# Autodesk Inventor assembly: Shipping goods QR subassembly 1 roq
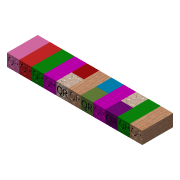
[picture p0: Inventor's stored thumbnail of the model, 180x180]
Saved by Autodesk Inventor 2015 (Build 190159000, 159)
## iProperties
Created: 2015-03-08
Part Number: Shipping goods QR subassembly 1 roq
Document SubType Name: Assembly
Designer: Vukica
Author: Vukica
## Documents named in this file (12)
- C:\Users\Vukica\Dropbox\IEEE\hardware rules\2016Hardware_Court_v6\Shipping goods QR subassembly 1 roq.iam
- C:\Users\Vukica\Dropbox\IEEE\hardware rules\2016Hardware_Court_v6\Container 2 2 5.ipt
- C:\Users\Vukica\Dropbox\IEEE\hardware rules\2016Hardware_Court_v6\Container 2 2 2 and half.ipt
- C:\Users\Vukica\Dropbox\IEEE\hardware rules\2016Hardware_Court_v6\Container 2 2 2 and half color 2.ipt
- C:\Users\Vukica\Dropbox\IEEE\hardware rules\2016Hardware_Court_v6\Container 2 2 2 and half color 4.ipt
- C:\Users\Vukica\Dropbox\IEEE\hardware rules\2016Hardware_Court_v6\Container 2 2 2 and half color 5.ipt
- C:\Users\Vukica\Dropbox\IEEE\hardware rules\2016Hardware_Court_v6\Container 2 2 2 and half color 7.ipt
- C:\Users\Vukica\Dropbox\IEEE\hardware rules\2016Hardware_Court_v6\Container 2 2 5 QR color 4.ipt
- C:\Users\Vukica\Dropbox\IEEE\hardware rules\2016Hardware_Court_v6\Container 2 2 5 QR color 5.ipt
- C:\Users\Vukica\Dropbox\IEEE\hardware rules\2016Hardware_Court_v6\Container 2 2 5 QR color 6.ipt
- C:\Users\Vukica\Dropbox\IEEE\hardware rules\2016Hardware_Court_v6\Container 2 2 5 QR color 1.ipt
- C:\Users\Vukica\Dropbox\IEEE\hardware rules\2016Hardware_Court_v6\Container 2 2 5 QR color 2.ipt
## Components (14 placed, 11 different names)
1. Container 2 2 5:1 — Flush:1, Mate:1, Flush:2, Flush:4, Mate:4, Flush:6, Flush:8
2. Container 2 2 2 and half:1 — Flush:1, Mate:1, Flush:2, Flush:3, Mate:2, Mate:8
3. Container 2 2 2 and half color 2:1 — Flush:5, Mate:3, Flush:7, Mate:5, Flush:9, Flush:10, Mate:9
4. Container 2 2 2 and half color 4:1 — Mate:7, Mate:8, Flush:13
5. Container 2 2 2 and half color 5:1 — Mate:9, Mate:10, Flush:14
6. Container 2 2 2 and half color 7:1 — Mate:13, Flush:19, Flush:20, Mate:14, Flush:21, Flush:22, Flush:23, Mate:32, Flush:56, Flush:57
7. Container 2 2 5 QR color 4:1 — Flush:3, Mate:2, Flush:4, Flush:5, Mate:3, Flush:7, Mate:7, Flush:13, Mate:10, Flush:14
8. Container 2 2 5 QR color 5:1 — Mate:6, Flush:11, Flush:12, Mate:11, Flush:15, Flush:16
9. Container 2 2 5 QR color 6:1 — Mate:11, Flush:15, Flush:16
10. Container 2 2 5 QR color 1:1 — Mate:5, Flush:9, Flush:10, Mate:13, Flush:19, Flush:20
11. Container 2 2 5 QR color 2:1 — Mate:4, Flush:6, Flush:8, Mate:6, Flush:11, Flush:12
12. Container 2 2 2 and half:2 — Mate:14, Flush:21, Flush:22, Flush:23
13. Container 2 2 5 QR color 2:4 — Mate:32, Flush:56, Flush:57, Mate:33, Flush:58, Flush:59
14. Container 2 2 5 QR color 4:3 — Mate:33, Flush:58, Flush:59
## Relationships (40: Flush 25, Mate 15)
- Flush:1: Container 2 2 5:1 ↔ Container 2 2 2 and half:1
- Mate:1: Container 2 2 5:1 ↔ Container 2 2 2 and half:1
- Flush:2: Container 2 2 5:1 ↔ Container 2 2 2 and half:1
- Flush:3: Container 2 2 2 and half:1 ↔ Container 2 2 5 QR color 4:1
- Mate:2: Container 2 2 2 and half:1 ↔ Container 2 2 5 QR color 4:1
- Flush:4: Container 2 2 5:1 ↔ Container 2 2 5 QR color 4:1
- Flush:5: Container 2 2 2 and half color 2:1 ↔ Container 2 2 5 QR color 4:1
- Mate:3: Container 2 2 2 and half color 2:1 ↔ Container 2 2 5 QR color 4:1
- Mate:4: Container 2 2 5:1 ↔ Container 2 2 5 QR color 2:1
- Flush:6: Container 2 2 5:1 ↔ Container 2 2 5 QR color 2:1
- Flush:7: Container 2 2 2 and half color 2:1 ↔ Container 2 2 5 QR color 4:1
- Flush:8: Container 2 2 5:1 ↔ Container 2 2 5 QR color 2:1
- Mate:5: Container 2 2 2 and half color 2:1 ↔ Container 2 2 5 QR color 1:1
- Flush:9: Container 2 2 2 and half color 2:1 ↔ Container 2 2 5 QR color 1:1
- Flush:10: Container 2 2 2 and half color 2:1 ↔ Container 2 2 5 QR color 1:1
- Mate:6: Container 2 2 5 QR color 5:1 ↔ Container 2 2 5 QR color 2:1
- Flush:11: Container 2 2 5 QR color 5:1 ↔ Container 2 2 5 QR color 2:1
- Flush:12: Container 2 2 5 QR color 5:1 ↔ Container 2 2 5 QR color 2:1
- Mate:7: Container 2 2 2 and half color 4:1 ↔ Container 2 2 5 QR color 4:1
- Mate:8: Container 2 2 2 and half:1 ↔ Container 2 2 2 and half color 4:1
- Flush:13: Container 2 2 2 and half color 4:1 ↔ Container 2 2 5 QR color 4:1
- Mate:9: Container 2 2 2 and half color 2:1 ↔ Container 2 2 2 and half color 5:1
- Mate:10: Container 2 2 2 and half color 5:1 ↔ Container 2 2 5 QR color 4:1
- Flush:14: Container 2 2 2 and half color 5:1 ↔ Container 2 2 5 QR color 4:1
- Mate:11: Container 2 2 5 QR color 5:1 ↔ Container 2 2 5 QR color 6:1
- Flush:15: Container 2 2 5 QR color 5:1 ↔ Container 2 2 5 QR color 6:1
- Flush:16: Container 2 2 5 QR color 5:1 ↔ Container 2 2 5 QR color 6:1
- Mate:13: Container 2 2 2 and half color 7:1 ↔ Container 2 2 5 QR color 1:1
- Flush:19: Container 2 2 2 and half color 7:1 ↔ Container 2 2 5 QR color 1:1
- Flush:20: Container 2 2 2 and half color 7:1 ↔ Container 2 2 5 QR color 1:1
- Mate:14: Container 2 2 2 and half color 7:1 ↔ Container 2 2 2 and half:2
- Flush:21: Container 2 2 2 and half color 7:1 ↔ Container 2 2 2 and half:2
- Flush:22: Container 2 2 2 and half color 7:1 ↔ Container 2 2 2 and half:2
- Flush:23: Container 2 2 2 and half color 7:1 ↔ Container 2 2 2 and half:2
- Mate:32: Container 2 2 2 and half color 7:1 ↔ Container 2 2 5 QR color 2:4
- Flush:56: Container 2 2 2 and half color 7:1 ↔ Container 2 2 5 QR color 2:4
- Flush:57: Container 2 2 2 and half color 7:1 ↔ Container 2 2 5 QR color 2:4
- Mate:33: Container 2 2 5 QR color 2:4 ↔ Container 2 2 5 QR color 4:3
- Flush:58: Container 2 2 5 QR color 2:4 ↔ Container 2 2 5 QR color 4:3
- Flush:59: Container 2 2 5 QR color 2:4 ↔ Container 2 2 5 QR color 4:3
